# Autodesk Inventor assembly: A_ankle_wing_001_MIR
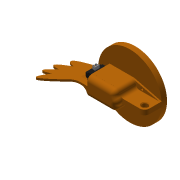
[picture p0: Inventor's stored thumbnail of the model, 180x180]
Saved by Autodesk Inventor 2016 (Build 200138000, 138)
## iProperties
Created: 2016-02-23
Part Number: A_ankle_wing_001_MIR
Document SubType Name: Assembly
Designer: Mateusz
Author: Mateusz
## Documents named in this file (9)
- D:\PROJECTS\2016_biped\hermes\mechanics_tmp\A_ankle_wing_001_MIR.iam
- D:\PROJECTS\2016_biped\hermes\mechanics_tmp\AX-12A.iam
- D:\PROJECTS\2016_biped\hermes\mechanics_tmp\P_ankle01_001.ipt
- D:\PROJECTS\2016_biped\hermes\mechanics_tmp\P_bearing_Z9089_001.ipt
- D:\PROJECTS\2016_biped\hermes\mechanics_tmp\P_ankle02_001_MIR.ipt
- D:\PROJECTS\2016_biped\hermes\mechanics_tmp\SharpIRsensor.ipt
- D:\PROJECTS\2016_biped\hermes\mechanics_tmp\P_ankle02front_001_MIR.ipt
- D:\PROJECTS\2016_biped\hermes\mechanics_tmp\P_akle02back_001_MIR.ipt
- D:\PROJECTS\2016_biped\hermes\mechanics_tmp\P_ankle03_001_MIR.ipt
## Components (8 placed, 8 different names)
1. AX-12A:1 [sub-assembly] — Mate:2, Angle:1, Mate:1, Mate:21, Mate:5, Mate:3, Angle:2
2. P_ankle01_001:1 — Mate:21, Mate:5, Mate:3, Flush:1, Mate:6, Tangent:1, Mate:8, Mate:21
3. P_bearing_Z9089_001:1 — Mate:7, Mate:6, Mate:21
4. P_ankle02_001_MIR:1 — Mate:13, Mate:12, Mate:11
5. SharpIRsensor:1 — Tangent:1, Mate:19, Mate:18
6. P_ankle02front_001_MIR:1 — Mate:17, Mate:10, Mate:8, Mate:22
7. P_akle02back_001_MIR:1 — Mate:19, Mate:18, Mate:16, Mate:15, Mate:14, Insert:1, Mate:20
8. P_ankle03_001_MIR:1 — Insert:1, Mate:20, Mate:22
## Relationships (26: Mate 20, Angle 2, Flush 2, Tangent 1, Insert 1)
- Mate:2: AX-12A:1
- Angle:1 (0 deg): AX-12A:1
- Mate:1: AX-12A:1
- Mate:21: AX-12A:1 ↔ P_ankle01_001:1
- Mate:5: AX-12A:1 ↔ P_ankle01_001:1
- Mate:3: AX-12A:1 ↔ P_ankle01_001:1
- Flush:1 [Mate]: P_ankle01_001:1
- Angle:2 (0 deg): AX-12A:1
- Mate:7: P_bearing_Z9089_001:1
- Mate:6: P_ankle01_001:1 ↔ P_bearing_Z9089_001:1
- Mate:13: P_ankle02_001_MIR:1
- Mate:12: P_ankle02_001_MIR:1
- Mate:11: P_ankle02_001_MIR:1
- Tangent:1: P_ankle01_001:1 ↔ SharpIRsensor:1
- Mate:17 [Flush]: P_ankle02front_001_MIR:1
- Mate:10: P_ankle02front_001_MIR:1
- Mate:8: P_ankle01_001:1 ↔ P_ankle02front_001_MIR:1
- Mate:19: SharpIRsensor:1 ↔ P_akle02back_001_MIR:1
- Mate:18: SharpIRsensor:1 ↔ P_akle02back_001_MIR:1
- Mate:16: P_akle02back_001_MIR:1
- Mate:15 [Flush]: P_akle02back_001_MIR:1
- Mate:14: P_akle02back_001_MIR:1
- Insert:1: P_akle02back_001_MIR:1 ↔ P_ankle03_001_MIR:1
- Mate:20: P_akle02back_001_MIR:1 ↔ P_ankle03_001_MIR:1
- Mate:21: P_ankle01_001:1 ↔ P_bearing_Z9089_001:1
- Mate:22: P_ankle02front_001_MIR:1 ↔ P_ankle03_001_MIR:1
